# Autodesk Inventor assembly: RSR25-880
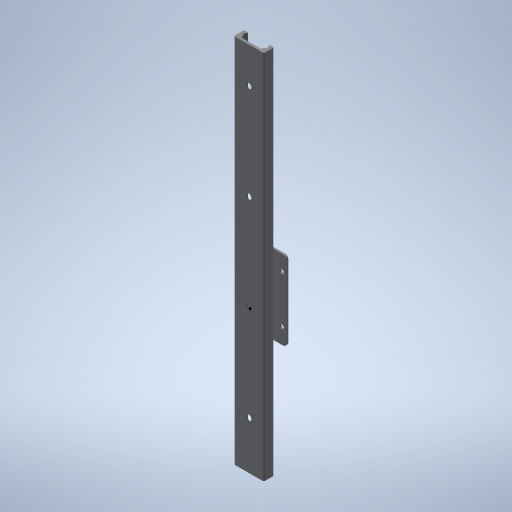
[picture p0: Inventor's stored thumbnail of the model, 512x512]
Saved by Autodesk Inventor 2024.1 (Build 281209000, 209)
## iProperties
Category: PARTsolutions
Company: MISUMI
Created: 2023-08-10
Part Number: RSR25-880
Catalog Web Link: www.cadenas.de
Description: RSR-Roller Slide Rails
Vendor: MISUMI
Document SubType Name: Assembly
Designer: psAdmin
Manufacturer: MISUMI
Mass: 87.9269 g
Surface Area: 779.784 cm^2
Volume: 87.9269 cm^3
PSOL_IDENT_0: {$CADENAS_DATA/23d-libs/misumi/metric/07_slide_rails/rsr_asmtab.prj},172 {VTYP=3D},{STYP=ASSTAB},{NB=
PSOL_IDENT_1: RSR25-880},{LINA=RSR25-880},{NN=RSR},{DATE=02.06.2021 03:22:41},{GEOMDATE=14.05.2012},{VERSION=},{LI
PSOL_IDENT_2: NEID=10},{WBVAR=LS,ALT,S},{WBNUMERIC=LS,S}  {NB=RSR25-880},{LINA=RSR25-880},{KT=DUMMY},{PN=RSR25-880
PSOL_IDENT_3: },{TYPE=RSR25},{MATR=Aluminum Alloy},{STR=Clear Anodizing},{MATS=304 Stainless Steel},{STS=-},{MATRO=
PSOL_IDENT_4: Polyacetal},{NO=25},{LS=880},{NH=11},{LL=40},{RM=176},{SM=40},{LS1=[160,240,320,400,480,560,640,720,
PSOL_IDENT_5: 800,880,960,1040,1200]},{T=RSRR},{PPATH=rsr_series/rsr_templ.prj},{ALT=},{S=0},{SALG=[0]}
NB: RSR25-880
NN: RSR
NT: Roller Slide Rails
NBSYN: $PN.
LINA: RSR25-880
CATALOG: Misumi
PN: RSR25-880
NO: 25
LS: 880
NH: 11
LL: 40
ALT: w/o Additional Sliders
S: 0
SUPPLIER: MISUMI
ARTICLENO: RSR25-880
BOMINFO: RSR25-880
CREATOR: CADENAS GmbH
Title: RSR25-880
Author: Cadenas PARTsolutions
Comments: Roller Slide Rails
## Documents named in this file (3)
- C:\Users\haruy\OneDrive - Kyushu University\KURT_工房共有\2023~2024\ハード\CAD\2024NHK\000_parts\スライダー\RSR25\RSR25-880\AIS2022\RSR25-880.iam
- C:\Users\haruy\OneDrive - Kyushu University\KURT_工房共有\2023~2024\ハード\CAD\2024NHK\000_parts\スライダー\RSR25\RSR25-880\AIS2022\RSRR25-880.ipt
- C:\Users\haruy\OneDrive - Kyushu University\KURT_工房共有\2023~2024\ハード\CAD\2024NHK\000_parts\スライダー\RSR25\RSR25-880\AIS2022\RSRS25.ipt
## Components (2 placed, 2 different names)
1. RSRR25-880:1 — to_slider_Z@1 <-> to_rail_Z@2, to_slider_YZ@1 <-> to_rail_YZ@2
2. RSRS25:1 — to_slider_Z@1 <-> to_rail_Z@2, to_slider_YZ@1 <-> to_rail_YZ@2
## Relationships (2: Mate 1, Angle 1)
- to_slider_Z@1 <-> to_rail_Z@2 [Mate]: RSRR25-880:1 ↔ RSRS25:1
- to_slider_YZ@1 <-> to_rail_YZ@2 [Angle] (180 deg): RSRR25-880:1 ↔ RSRS25:1
